# Autodesk Inventor assembly: ballRampWithStepForBallLeftSide
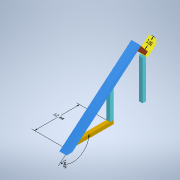
[picture p0: Inventor's stored thumbnail of the model, 180x180]
Saved by Autodesk Inventor 2020.2 (Build 242310000, 310)
## iProperties
Created: 2020-01-26
Part Number: ballRampWithStepForBallLeftSide
Document SubType Name: Assembly
Designer: robst
Author: robst
## Documents named in this file (9)
- C:\git\CAD-Development\robSteele\2020CompetitionRobot\ballRampWithStepForBallLeftSide.iam
- C:\git\CAD-Development\robSteele\2020CompetitionRobot\Aluminum1x1Base.ipt
- C:\git\CAD-Development\robSteele\2020CompetitionRobot\Aluminum1x2HypotLowerPortion.ipt
- C:\git\CAD-Development\robSteele\2020CompetitionRobot\Aluminum1x2Step.ipt
- C:\git\CAD-Development\robSteele\2020CompetitionRobot\Aluminum1x2HypotTop.ipt
- C:\git\CAD-Development\robSteele\2020CompetitionRobot\Aluminum1x1MiddleFront.ipt
- C:\git\CAD-Development\robSteele\2020CompetitionRobot\Aluminum1x1MiddleBack.ipt
- C:\git\CAD-Development\robSteele\2020CompetitionRobot\40-50-6in-Template.ipt
- C:\git\CAD-Development\robSteele\2020CompetitionRobot\rectangular3_5x5_0-in-Template.ipt
## Components (10 placed, 8 different names)
1. Aluminum1x1Base:1 — Flush:2, Mate:5, Mate:8, Flush:10, Mate:10, Flush:13, Mate:17, Flush:16, Flush:20, Mate:19, Mate:20, Flush:21, Flush:22, Mate:21, Flush:23
2. Aluminum1x2HypotLowerPortion:1 — Flush:2, Mate:5, Mate:11, Mate:13, Flush:17, Mate:18, Flush:18, Flush:19, Flush:20
3. Aluminum1x2Step:1 — Mate:3, Flush:5, Flush:6, Flush:12, Mate:18, Flush:18, Flush:19
4. Aluminum1x2HypotTop:1 — Mate:3, Flush:5, Flush:6, Flush:11, Mate:14
5. Aluminum1x1MiddleFront:1 — Mate:20, Flush:21, Flush:22, Mate:22
6. Aluminum1x1MiddleBack:1 — Mate:8, Flush:10, Mate:19, Mate:21, Flush:23, Mate:22
7. 40-50-6in-Template:1 — Mate:10, Mate:11, Flush:13
8. 40-50-6in-Template:2 — Mate:13
9. 40-50-6in-Template:3 — Mate:14
10. rectangular3_5x5_0-in-Template:1 — Mate:17, Flush:16
## Relationships (28: Flush 15, Mate 13)
- Flush:2: Aluminum1x1Base:1 ↔ Aluminum1x2HypotLowerPortion:1
- Mate:3: Aluminum1x2Step:1 ↔ Aluminum1x2HypotTop:1
- Flush:5: Aluminum1x2Step:1 ↔ Aluminum1x2HypotTop:1
- Flush:6: Aluminum1x2Step:1 ↔ Aluminum1x2HypotTop:1
- Mate:5: Aluminum1x1Base:1 ↔ Aluminum1x2HypotLowerPortion:1
- Mate:8: Aluminum1x1Base:1 ↔ Aluminum1x1MiddleBack:1
- Flush:10: Aluminum1x1Base:1 ↔ Aluminum1x1MiddleBack:1
- Flush:11 (88.9 mm): Aluminum1x2HypotTop:1
- Flush:12 (88.9 mm): Aluminum1x2Step:1
- Mate:10: Aluminum1x1Base:1 ↔ 40-50-6in-Template:1
- Mate:11: Aluminum1x2HypotLowerPortion:1 ↔ 40-50-6in-Template:1
- Flush:13: Aluminum1x1Base:1 ↔ 40-50-6in-Template:1
- Mate:13: Aluminum1x2HypotLowerPortion:1 ↔ 40-50-6in-Template:2
- Mate:14: Aluminum1x2HypotTop:1 ↔ 40-50-6in-Template:3
- Mate:17: Aluminum1x1Base:1 ↔ rectangular3_5x5_0-in-Template:1
- Flush:16: Aluminum1x1Base:1 ↔ rectangular3_5x5_0-in-Template:1
- Flush:17 (76.2 mm): Aluminum1x2HypotLowerPortion:1
- Mate:18: Aluminum1x2HypotLowerPortion:1 ↔ Aluminum1x2Step:1
- Flush:18: Aluminum1x2HypotLowerPortion:1 ↔ Aluminum1x2Step:1
- Flush:19: Aluminum1x2HypotLowerPortion:1 ↔ Aluminum1x2Step:1
- Flush:20: Aluminum1x1Base:1 ↔ Aluminum1x2HypotLowerPortion:1
- Mate:19: Aluminum1x1Base:1 ↔ Aluminum1x1MiddleBack:1
- Mate:20: Aluminum1x1Base:1 ↔ Aluminum1x1MiddleFront:1
- Flush:21: Aluminum1x1Base:1 ↔ Aluminum1x1MiddleFront:1
- Flush:22: Aluminum1x1Base:1 ↔ Aluminum1x1MiddleFront:1
- Mate:21: Aluminum1x1Base:1 ↔ Aluminum1x1MiddleBack:1
- Flush:23: Aluminum1x1Base:1 ↔ Aluminum1x1MiddleBack:1
- Mate:22 (203.2 mm): Aluminum1x1MiddleFront:1 ↔ Aluminum1x1MiddleBack:1
